# Autodesk Inventor assembly: Alpha Motor Assembly
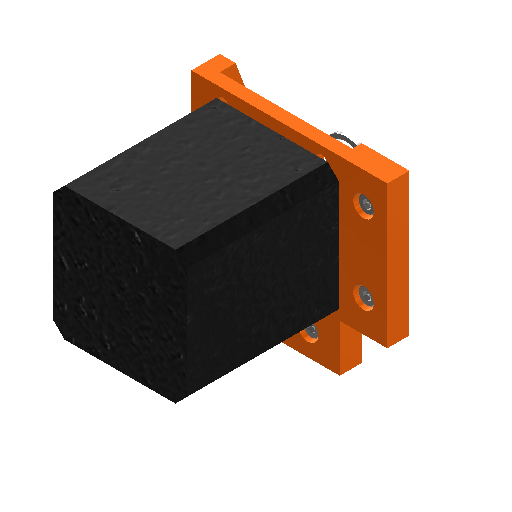
[picture p0: Inventor's stored thumbnail of the model, 512x512]
Saved by Autodesk Inventor 2023.2 (Build 272271000, 271)
## iProperties
Created: 2023-02-03
Part Number: Alpha Motor Assembly
Document SubType Name: Assembly
Designer: remop
Author: remop
## Documents named in this file (5)
- C:\Users\remop\OneDrive\Documents\Inventor\3D Printers\LuEVO\Mk5_FullKinematic\Alpha Motor Assembly.iam
- C:\Users\remop\OneDrive\Documents\Inventor\3D Printers\LuEVO\Mk5_FullKinematic\Alpha Motor Mount.ipt
- C:\Users\remop\OneDrive\Documents\Inventor\3D Printers\LuEVO\Mk5_FullKinematic\XY Axis Motor (Stepper).ipt
- C:\Users\remop\OneDrive\Documents\Inventor\3D Printers\LuEVO\Mk1\Belt_Pulley_20T.ipt
- C:\Users\remop\OneDrive\Documents\Inventor\Content Center Files\R2023\en-US\AS 1420\AS 1420 - 1973 - M3 x 6.ipt
## Components (12 placed, 4 different names)
1. Alpha Motor Mount:1 — Rigid:1, Insert:5, Insert:7, Insert:9, Insert:11, Insert:12, Insert:13, Insert:14, Insert:15, Insert:16
2. XY Axis Motor (Stepper):1 — Rigid:1, Rigid:2
3. Belt_Pulley_20T:1 — Rigid:2
4. AS 1420 - Metric M3 x 6:4 — Insert:5
5. AS 1420 - Metric M3 x 6:6 — Insert:7
6. AS 1420 - Metric M3 x 6:8 — Insert:9
7. AS 1420 - Metric M3 x 6:10 — Insert:11
8. AS 1420 - Metric M3 x 6:11 — Insert:12
9. AS 1420 - Metric M3 x 6:12 — Insert:13
10. AS 1420 - Metric M3 x 6:13 — Insert:14
11. AS 1420 - Metric M3 x 6:14 — Insert:15
12. AS 1420 - Metric M3 x 6:15 — Insert:16
## Relationships (11: Insert 9, WeldJoint 2)
- Rigid:1 [WeldJoint]: Alpha Motor Mount:1 ↔ XY Axis Motor (Stepper):1
- Rigid:2 [WeldJoint] (-0.5 mm): XY Axis Motor (Stepper):1 ↔ Belt_Pulley_20T:1
- Insert:5: Alpha Motor Mount:1 ↔ AS 1420 - Metric M3 x 6:4
- Insert:7: Alpha Motor Mount:1 ↔ AS 1420 - Metric M3 x 6:6
- Insert:9: Alpha Motor Mount:1 ↔ AS 1420 - Metric M3 x 6:8
- Insert:11: Alpha Motor Mount:1 ↔ AS 1420 - Metric M3 x 6:10
- Insert:12: Alpha Motor Mount:1 ↔ AS 1420 - Metric M3 x 6:11
- Insert:13: Alpha Motor Mount:1 ↔ AS 1420 - Metric M3 x 6:12
- Insert:14: Alpha Motor Mount:1 ↔ AS 1420 - Metric M3 x 6:13
- Insert:15: Alpha Motor Mount:1 ↔ AS 1420 - Metric M3 x 6:14
- Insert:16: Alpha Motor Mount:1 ↔ AS 1420 - Metric M3 x 6:15
